# Autodesk Inventor assembly: canard_assemb3
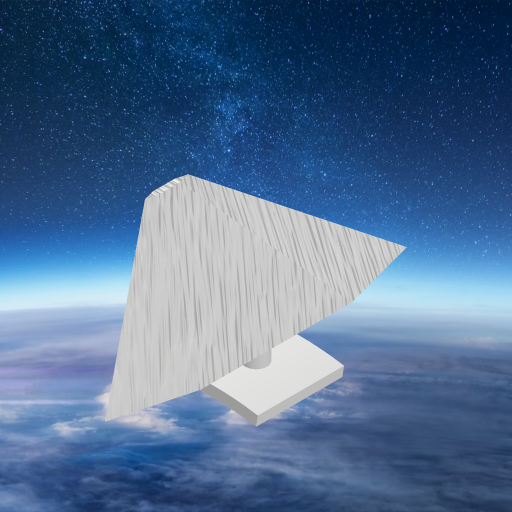
[picture p0: Inventor's stored thumbnail of the model, 512x512]
Saved by Autodesk Inventor 2023 (Build 270158000, 158)
## iProperties
Created: 2023-10-24
Part Number: canard_assemb3
Document SubType Name: Assembly
Designer: 310611102
Author: 310611102
## Documents named in this file (3)
- C:\Users\310611102\Documents\Inventor\SSR\avionics_2023ver\assembly\canard_assemb3.iam
- C:\Users\310611102\Documents\Inventor\SSR\avionics_2023ver\actuator_system\shiftt_fixed_plate2.ipt
- C:\Users\310611102\Documents\Inventor\SSR\avionics_2023ver\actuator_system\canard.ipt
## Components (2 placed, 2 different names)
1. shiftt_fixed_plate2:1 — Insert:1, Cylindrical:1
2. canard:1 — Insert:1, Cylindrical:1
## Relationships (2: Insert 1, CylindricalJoint 1)
- Insert:1: shiftt_fixed_plate2:1 ↔ canard:1
- Cylindrical:1: shiftt_fixed_plate2:1 ↔ canard:1
